# Autodesk Inventor assembly: Wheel
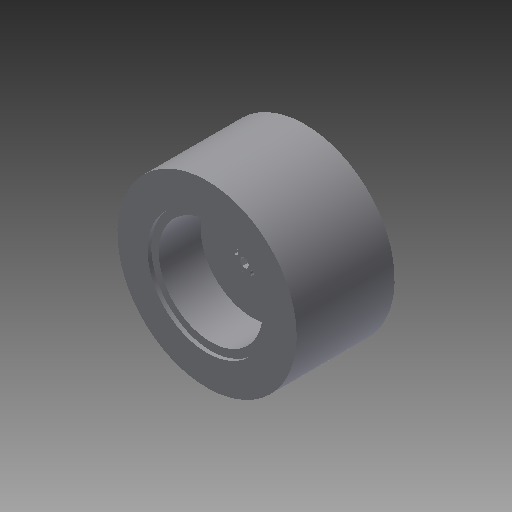
[picture p0: Inventor's stored thumbnail of the model, 512x512]
Saved by Autodesk Inventor 2019 (Build 230136000, 136)
## iProperties
Created: 2019-03-02
Part Number: Wheel
Document SubType Name: Assembly
Designer: alarr
Author: alarr
## Documents named in this file (3)
- C:\Users\alarr\OneDrive\Documents\Inventor\Mr.Green\Wheel.iam
- C:\Users\alarr\OneDrive\Documents\Inventor\Mr.Green\Wheel_Rim.ipt
- C:\Users\alarr\OneDrive\Documents\Inventor\Mr.Green\Wheel_Tire.ipt
## Components (2 placed, 2 different names)
1. Wheel_Rim:1 — Flush:1
2. Wheel_Tire:1 — Flush:1
## Relationships (1: Flush 1)
- Flush:1: Wheel_Rim:1 ↔ Wheel_Tire:1
